# Autodesk Inventor assembly: Gehäuse komplett
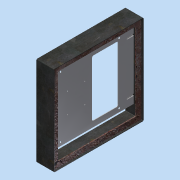
[picture p0: Inventor's stored thumbnail of the model, 180x180]
Saved by Autodesk Inventor 2015 SP1 (Build 190203100, 203)
## iProperties
Created: 2015-04-14
Part Number: Gehäuse komplett
Document SubType Name: Assembly
Designer: ElMatinho
Author: ElMatinho
## Documents named in this file (4)
- D:\FÜP\Gehäuse komplett.iam
- D:\FÜP\Aussengehäuse.ipt
- D:\FÜP\Frontplatte.ipt
- D:\FÜP\Innengehäuse gebogen.ipt
## Components (3 placed, 3 different names)
1. Aussengehäuse:1 — Fluchtend:1, Passend:1, Passend:2, Passend:3, Fluchtend:2, Passend:4
2. Frontplatte:1 — Fluchtend:1, Passend:1, Passend:2
3. Innengehäuse gebogen:1 — Passend:3, Fluchtend:2, Passend:4
## Relationships (6: Mate 4, Flush 2)
- Fluchtend:1 [Flush] (5 mm): Aussengehäuse:1 ↔ Frontplatte:1
- Passend:1 [Mate]: Aussengehäuse:1 ↔ Frontplatte:1
- Passend:2 [Mate]: Aussengehäuse:1 ↔ Frontplatte:1
- Passend:3 [Mate] (0.5 mm): Aussengehäuse:1 ↔ Innengehäuse gebogen:1
- Fluchtend:2 [Flush]: Aussengehäuse:1 ↔ Innengehäuse gebogen:1
- Passend:4 [Mate] (29.5 mm): Aussengehäuse:1 ↔ Innengehäuse gebogen:1
